# Autodesk Inventor assembly: 4x2 Angle
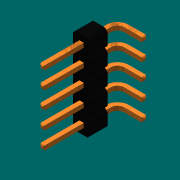
[picture p0: Inventor's stored thumbnail of the model, 180x180]
Saved by Autodesk Inventor 2016 SP1 (Build 200210100, 210)
## iProperties
Created: 2014-10-19
Part Number: 4x2 Angle
Document SubType Name: Assembly
Designer: Sawaiz Syed
Author: Sawaiz Syed
## Documents named in this file (2)
- C:\Users\sawai\OneDrive\projects\mppcInterface\cad\connector\2.54Header\rightAngle\1x5Angle.iam
- C:\Users\sawai\OneDrive\projects\mppcInterface\cad\connector\2.54Header\rightAngle\1x1Angle.iam
## Components (5 placed, 1 different names)
1. 1x1Angle:1 [sub-assembly]
2. 1x1Angle:2 [sub-assembly]
3. 1x1Angle:3 [sub-assembly]
4. 1x1Angle:4 [sub-assembly]
5. 1x1Angle:5 [sub-assembly]
## Component patterns: (5 elements, first: 1x1Angle:1)
